# Autodesk Inventor assembly: one roller asmb
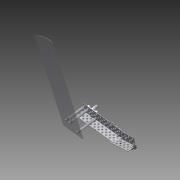
[picture p0: Inventor's stored thumbnail of the model, 180x180]
Saved by Autodesk Inventor 2014 SP1 (Build 180222100, 222)
## iProperties
Created: 2014-03-20
Part Number: one roller asmb
Document SubType Name: Assembly
Designer: Ryan
Author: Ryan
## Documents named in this file (14)
- C:\Users\Ryan\Desktop\sw\toss up 5th A bot\intake\plate attachment .iam
- C:\Users\Ryan\Desktop\sw\lib\Aperture VEX CAD Library\Metal\L Bar\2 x 5.ipt
- C:\Users\Ryan\Desktop\sw\lib\Aperture VEX CAD Library\Hardware\8-32\8-32_.375.ipt
- C:\Users\Ryan\Desktop\sw\lib\Aperture VEX CAD Library\Hardware\8-32\8-32 nylock.ipt
- C:\Users\Ryan\Desktop\sw\lib\Aperture VEX CAD Library\Metal\Custom 1 bar\5.ipt
- C:\Users\Ryan\Desktop\sw\lib\Aperture VEX CAD Library\Bearing Blocks\Bearing Block.ipt
- C:\Users\Ryan\Desktop\sw\lib\Aperture VEX CAD Library\Hardware\8-32\8-32_.250.ipt
- C:\Users\Ryan\Desktop\sw\lib\Aperture VEX CAD Library\Standoffs\BEAM-0500.ipt
- C:\Users\Ryan\Desktop\sw\lib\Aperture VEX CAD Library\Standoffs\BEAM-2000.ipt
- C:\Users\Ryan\Desktop\sw\lib\Aperture VEX CAD Library\Hardware\8-32\8-23_.750.ipt
- C:\Users\Ryan\Desktop\sw\lib\Aperture VEX CAD Library\Spacers\SPACER-0500-0125.ipt
- C:\Users\Ryan\Desktop\sw\lib\Aperture VEX CAD Library\Spacers\SPACER-0500-0375.ipt
- C:\Users\Ryan\Desktop\sw\lib\Aperture VEX CAD Library\Metal\L Bar\2 x 10.ipt
- C:\Users\Ryan\Desktop\sw\toss up 5th A bot\intake\large ball holder.ipt
## Components (36 placed, 13 different names)
1. 2 x 5:2 — Mate:28, Mate:29, Mate:30, Mate:31, Mate:36, Mate:37, Mate:38, Mate:44, Mate:64, Mate:65, Mate:66, Mate:67, Mate:68, Mate:69, Mate:70, Flush:1
2. 2 x 10:1 — Mate:31, Mate:32, Mate:33, Mate:35, Mate:45, Mate:46, Mate:51, Mate:59, Mate:60, Mate:62, Mate:83, Mate:86, Mate:90, Mate:91, Mate:92, Mate:95, Mate:96, Mate:97
3. 8-32_.375:5 — Mate:28, Mate:29, Mate:30, Mate:32, Mate:33, Mate:34
4. 8-32 nylock:5 — Mate:34, Mate:35
5. 5:1 — Mate:36, Mate:41, Mate:42, Mate:43, Mate:47, Mate:48, Mate:49
6. 8-32_.375:6 — Mate:37, Mate:38, Mate:40, Mate:41, Mate:42, Mate:43
7. 8-32 nylock:6 — Mate:40, Mate:44
8. 8-32_.375:7 — Mate:45, Mate:46, Mate:47, Mate:48, Mate:49, Mate:50
9. 8-32 nylock:7 — Mate:50, Mate:51
10. Bearing Block:2 — Mate:56, Mate:57, Mate:58, Mate:59, Mate:62, Mate:86, Mate:87
11. Bearing Block:3 — Mate:56, Mate:57, Mate:58, Mate:60, Mate:88, Mate:102, Mate:103
12. 8-32_.250:1 — Mate:68, Mate:69, Mate:70, Mate:71
13. BEAM-0500:1 — Mate:71, Flush:1
14. BEAM-2000:4 — Mate:98, Mate:99
15. 8-32 nylock:17 — Mate:95, Mate:96, Mate:97
16. 8-32 nylock:18 — Mate:98, Mate:99, Mate:106, Mate:107, Mate:111
17. SPACER-0500-0125:1 — Mate:102, Mate:103, Mate:104, Mate:105
18. SPACER-0500-0375:1 — Mate:104, Mate:105
19. 8-32_.375:10 — Mate:106, Mate:107, Mate:112
20. large ball holder:1 — Mate:111, Mate:112, Mate:113
21. 8-32 nylock:9 — Mate:63, Mate:67
22. 8-32_.375:8 — Mate:63, Mate:64, Mate:65, Mate:66
23. 8-32 nylock:10
24. 8-32_.375:9
25. 8-23_.750:2 — Mate:87, Mate:88, Mate:89
26. 8-32 nylock:14 — Mate:89, Mate:90
27. 8-23_.750:3
28. 8-32 nylock:15
29. BEAM-2000:2 — Mate:84, Mate:85, Mate:100, Mate:101
30. 8-32 nylock:12 — Mate:83, Mate:84, Mate:85, Mate:91, Mate:92
31. 8-32 nylock:20 — Mate:100, Mate:101, Mate:108, Mate:109
32. 8-32_.375:11 — Mate:108, Mate:109
33. BEAM-2000:3
34. 8-32 nylock:16
35. 8-32 nylock:21
36. 8-32_.375:12 — Mate:113
## Component patterns: (2 elements, first: 8-32 nylock:9 + 8-32_.375:8), (2 elements, first: 8-23_.750:2 + 8-32 nylock:14), (2 elements, first: BEAM-2000:2 + 8-32 nylock:12 + 8-32 nylock:20 + 8-32_.375:11)
## Relationships (69: Mate 68, Flush 1)
- Mate:28: 2 x 5:2 ↔ 8-32_.375:5
- Mate:29 (2.3114 mm): 2 x 5:2 ↔ 8-32_.375:5
- Mate:30 (2.3114 mm): 2 x 5:2 ↔ 8-32_.375:5
- Mate:31: 2 x 5:2 ↔ 2 x 10:1
- Mate:32 (2.3114 mm): 2 x 10:1 ↔ 8-32_.375:5
- Mate:33 (2.3114 mm): 2 x 10:1 ↔ 8-32_.375:5
- Mate:34: 8-32_.375:5 ↔ 8-32 nylock:5
- Mate:35: 2 x 10:1 ↔ 8-32 nylock:5
- Mate:36: 2 x 5:2 ↔ 5:1
- Mate:37 (2.3114 mm): 2 x 5:2 ↔ 8-32_.375:6
- Mate:38 (2.3114 mm): 2 x 5:2 ↔ 8-32_.375:6
- Mate:40: 8-32_.375:6 ↔ 8-32 nylock:6
- Mate:41 (2.3114 mm): 5:1 ↔ 8-32_.375:6
- Mate:42 (2.3114 mm): 5:1 ↔ 8-32_.375:6
- Mate:43: 5:1 ↔ 8-32_.375:6
- Mate:44: 2 x 5:2 ↔ 8-32 nylock:6
- Mate:45 (2.3114 mm): 2 x 10:1 ↔ 8-32_.375:7
- Mate:46 (2.3114 mm): 2 x 10:1 ↔ 8-32_.375:7
- Mate:47 (2.3114 mm): 5:1 ↔ 8-32_.375:7
- Mate:48 (2.3114 mm): 5:1 ↔ 8-32_.375:7
- Mate:49: 5:1 ↔ 8-32_.375:7
- Mate:50: 8-32_.375:7 ↔ 8-32 nylock:7
- Mate:51: 2 x 10:1 ↔ 8-32 nylock:7
- Mate:56: Bearing Block:2 ↔ Bearing Block:3
- Mate:57: Bearing Block:2 ↔ Bearing Block:3
- Mate:58: Bearing Block:2 ↔ Bearing Block:3
- Mate:59: 2 x 10:1 ↔ Bearing Block:2
- Mate:60 (-23.0886 mm): 2 x 10:1 ↔ Bearing Block:3
- Mate:62 (27.7114 mm): 2 x 10:1 ↔ Bearing Block:2
- Mate:63: 8-32 nylock:9 ↔ 8-32_.375:8
- Mate:64: 2 x 5:2 ↔ 8-32_.375:8
- Mate:65 (2.3114 mm): 2 x 5:2 ↔ 8-32_.375:8
- Mate:66 (2.3114 mm): 2 x 5:2 ↔ 8-32_.375:8
- Mate:67 (1.1684 mm): 2 x 5:2 ↔ 8-32 nylock:9
- Mate:68 (15.0114 mm): 2 x 5:2 ↔ 8-32_.250:1
- Mate:69 (1.1684 mm): 2 x 5:2 ↔ 8-32_.250:1
- Mate:70 (2.3114 mm): 2 x 5:2 ↔ 8-32_.250:1
- Mate:71: 8-32_.250:1 ↔ BEAM-0500:1
- Flush:1: 2 x 5:2 ↔ BEAM-0500:1
- Mate:83: 2 x 10:1 ↔ 8-32 nylock:12
- Mate:84: BEAM-2000:2 ↔ 8-32 nylock:12
- Mate:85: BEAM-2000:2 ↔ 8-32 nylock:12
- Mate:86 (2.3114 mm): 2 x 10:1 ↔ Bearing Block:2
- Mate:87: Bearing Block:2 ↔ 8-23_.750:2
- Mate:88: Bearing Block:3 ↔ 8-23_.750:2
- Mate:89: 8-23_.750:2 ↔ 8-32 nylock:14
- Mate:90: 2 x 10:1 ↔ 8-32 nylock:14
- Mate:91 (2.3114 mm): 2 x 10:1 ↔ 8-32 nylock:12
- Mate:92 (-23.0886 mm): 2 x 10:1 ↔ 8-32 nylock:12
- [Mate]: BEAM-2000:4 ↔ 8-32 nylock:17
- [Mate]: BEAM-2000:4 ↔ 8-32 nylock:17
- Mate:95 (2.3114 mm): 2 x 10:1 ↔ 8-32 nylock:17
- Mate:96 (-23.0886 mm): 2 x 10:1 ↔ 8-32 nylock:17
- Mate:97: 2 x 10:1 ↔ 8-32 nylock:17
- Mate:98: BEAM-2000:4 ↔ 8-32 nylock:18
- Mate:99: BEAM-2000:4 ↔ 8-32 nylock:18
- Mate:100: BEAM-2000:2 ↔ 8-32 nylock:20
- Mate:101: BEAM-2000:2 ↔ 8-32 nylock:20
- Mate:102: Bearing Block:3 ↔ SPACER-0500-0125:1
- Mate:103: Bearing Block:3 ↔ SPACER-0500-0125:1
- Mate:104: SPACER-0500-0125:1 ↔ SPACER-0500-0375:1
- Mate:105: SPACER-0500-0125:1 ↔ SPACER-0500-0375:1
- Mate:106: 8-32 nylock:18 ↔ 8-32_.375:10
- Mate:107 (1.5875 mm): 8-32 nylock:18 ↔ 8-32_.375:10
- Mate:108: 8-32 nylock:20 ↔ 8-32_.375:11
- Mate:109 (1.5875 mm): 8-32 nylock:20 ↔ 8-32_.375:11
- Mate:111: 8-32 nylock:18 ↔ large ball holder:1
- Mate:112: 8-32_.375:10 ↔ large ball holder:1
- Mate:113: large ball holder:1 ↔ 8-32_.375:12
## Named parameters: q = 2.3114 mm, d178_d160 = 0 mm, d179_d161 = 0 mm
